(part 1 of 2)
# Autodesk Inventor assembly: Shield_99
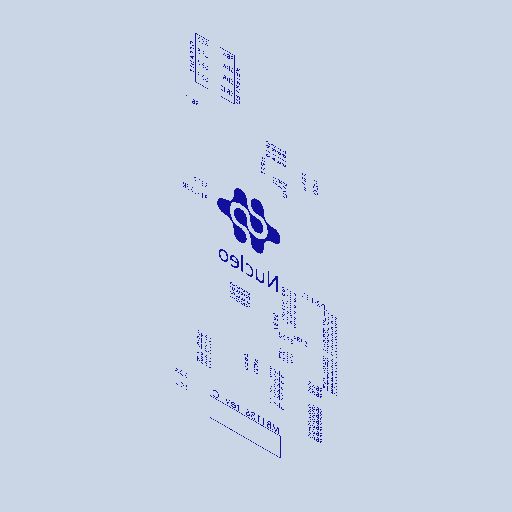
[picture p0: Inventor's stored thumbnail of the model, 512x512]
Saved by Autodesk Inventor 2022 (Build 260153000, 153)
## iProperties
Created: 2022-03-24
Part Number: Shield_99
Document SubType Name: Assembly
Designer: dvorakj
Author: dvorakj
## Documents named in this file (319)
- C:\Users\dvorakj\Documents\Inventor\Bakalarka\altium export\Shield_99.iam
- C:\Users\dvorakj\Documents\Inventor\Bakalarka\altium export\NUCLEO-F411RE_PCB_BOTTOM_Overlay_Varsay_X_8Dlan.ipt
- C:\Users\dvorakj\Documents\Inventor\Bakalarka\altium export\NUCLEO-F411RE_PCB_BOTTOM_Overlay_Varsay_X_8Dlan_1.ipt
- C:\Users\dvorakj\Documents\Inventor\Bakalarka\altium export\NUCLEO-F411RE_PCB_BOTTOM_Overlay_Varsay_X_8Dlan_2.ipt
- C:\Users\dvorakj\Documents\Inventor\Bakalarka\altium export\NUCLEO-F411RE_PCB_BOTTOM_Overlay_Varsay_X_8Dlan_3.ipt
- C:\Users\dvorakj\Documents\Inventor\Bakalarka\altium export\NUCLEO-F411RE_PCB_BOTTOM_Overlay_Varsay_X_8Dlan_4.ipt
- C:\Users\dvorakj\Documents\Inventor\Bakalarka\altium export\NUCLEO-F411RE_PCB_BOTTOM_Overlay_Varsay_X_8Dlan_5.ipt
- C:\Users\dvorakj\Documents\Inventor\Bakalarka\altium export\NUCLEO-F411RE_PCB_BOTTOM_Overlay_Varsay_X_8Dlan_6.ipt
- C:\Users\dvorakj\Documents\Inventor\Bakalarka\altium export\NUCLEO-F411RE_PCB_BOTTOM_Overlay_Varsay_X_8Dlan_7.ipt
- C:\Users\dvorakj\Documents\Inventor\Bakalarka\altium export\NUCLEO-F411RE_PCB_BOTTOM_Overlay_Varsay_X_8Dlan_8.ipt
- C:\Users\dvorakj\Documents\Inventor\Bakalarka\altium export\NUCLEO-F411RE_PCB_BOTTOM_Overlay_Varsay_X_8Dlan_9.ipt
- C:\Users\dvorakj\Documents\Inventor\Bakalarka\altium export\NUCLEO-F411RE_PCB_BOTTOM_Overlay_Varsay_X_8Dlan_10.ipt
- C:\Users\dvorakj\Documents\Inventor\Bakalarka\altium export\NUCLEO-F411RE_PCB_BOTTOM_Overlay_Varsay_X_8Dlan_11.ipt
- C:\Users\dvorakj\Documents\Inventor\Bakalarka\altium export\NUCLEO-F411RE_PCB_BOTTOM_Overlay_Varsay_X_8Dlan_12.ipt
- C:\Users\dvorakj\Documents\Inventor\Bakalarka\altium export\NUCLEO-F411RE_PCB_BOTTOM_Overlay_Varsay_X_8Dlan_13.ipt
- C:\Users\dvorakj\Documents\Inventor\Bakalarka\altium export\NUCLEO-F411RE_PCB_BOTTOM_Overlay_Varsay_X_8Dlan_14.ipt
- C:\Users\dvorakj\Documents\Inventor\Bakalarka\altium export\NUCLEO-F411RE_PCB_BOTTOM_Overlay_Varsay_X_8Dlan_15.ipt
- C:\Users\dvorakj\Documents\Inventor\Bakalarka\altium export\NUCLEO-F411RE_PCB_BOTTOM_Overlay_Varsay_X_8Dlan_16.ipt
- C:\Users\dvorakj\Documents\Inventor\Bakalarka\altium export\NUCLEO-F411RE_PCB_BOTTOM_Overlay_Varsay_X_8Dlan_17.ipt
- C:\Users\dvorakj\Documents\Inventor\Bakalarka\altium export\NUCLEO-F411RE_PCB_BOTTOM_Overlay_Varsay_X_8Dlan_18.ipt
- C:\Users\dvorakj\Documents\Inventor\Bakalarka\altium export\NUCLEO-F411RE_PCB_BOTTOM_Overlay_Varsay_X_8Dlan_19.ipt
- C:\Users\dvorakj\Documents\Inventor\Bakalarka\altium export\NUCLEO-F411RE_PCB_BOTTOM_Overlay_Varsay_X_8Dlan_20.ipt
- C:\Users\dvorakj\Documents\Inventor\Bakalarka\altium export\NUCLEO-F411RE_PCB_BOTTOM_Overlay_Varsay_X_8Dlan_21.ipt
- C:\Users\dvorakj\Documents\Inventor\Bakalarka\altium export\NUCLEO-F411RE_PCB_BOTTOM_Overlay_Varsay_X_8Dlan_22.ipt
- C:\Users\dvorakj\Documents\Inventor\Bakalarka\altium export\NUCLEO-F411RE_PCB_BOTTOM_Overlay_Varsay_X_8Dlan_23.ipt
- C:\Users\dvorakj\Documents\Inventor\Bakalarka\altium export\NUCLEO-F411RE_PCB_BOTTOM_Overlay_Varsay_X_8Dlan_24.ipt
- C:\Users\dvorakj\Documents\Inventor\Bakalarka\altium export\NUCLEO-F411RE_PCB_BOTTOM_Overlay_Varsay_X_8Dlan_25.ipt
- C:\Users\dvorakj\Documents\Inventor\Bakalarka\altium export\NUCLEO-F411RE_PCB_BOTTOM_Overlay_Varsay_X_8Dlan_26.ipt
- C:\Users\dvorakj\Documents\Inventor\Bakalarka\altium export\NUCLEO-F411RE_PCB_BOTTOM_Overlay_Varsay_X_8Dlan_27.ipt
- C:\Users\dvorakj\Documents\Inventor\Bakalarka\altium export\NUCLEO-F411RE_PCB_BOTTOM_Overlay_Varsay_X_8Dlan_28.ipt
- C:\Users\dvorakj\Documents\Inventor\Bakalarka\altium export\NUCLEO-F411RE_PCB_BOTTOM_Overlay_Varsay_X_8Dlan_29.ipt
- C:\Users\dvorakj\Documents\Inventor\Bakalarka\altium export\NUCLEO-F411RE_PCB_BOTTOM_Overlay_Varsay_X_8Dlan_30.ipt
- C:\Users\dvorakj\Documents\Inventor\Bakalarka\altium export\NUCLEO-F411RE_PCB_BOTTOM_Overlay_Varsay_X_8Dlan_31.ipt
- C:\Users\dvorakj\Documents\Inventor\Bakalarka\altium export\NUCLEO-F411RE_PCB_BOTTOM_Overlay_Varsay_X_8Dlan_32.ipt
- C:\Users\dvorakj\Documents\Inventor\Bakalarka\altium export\NUCLEO-F411RE_PCB_BOTTOM_Overlay_Varsay_X_8Dlan_33.ipt
- C:\Users\dvorakj\Documents\Inventor\Bakalarka\altium export\NUCLEO-F411RE_PCB_BOTTOM_Overlay_Varsay_X_8Dlan_34.ipt
- C:\Users\dvorakj\Documents\Inventor\Bakalarka\altium export\NUCLEO-F411RE_PCB_BOTTOM_Overlay_Varsay_X_8Dlan_35.ipt
- C:\Users\dvorakj\Documents\Inventor\Bakalarka\altium export\NUCLEO-F411RE_PCB_BOTTOM_Overlay_Varsay_X_8Dlan_36.ipt
- C:\Users\dvorakj\Documents\Inventor\Bakalarka\altium export\NUCLEO-F411RE_PCB_BOTTOM_Overlay_Varsay_X_8Dlan_37.ipt
- C:\Users\dvorakj\Documents\Inventor\Bakalarka\altium export\NUCLEO-F411RE_PCB_BOTTOM_Overlay_Varsay_X_8Dlan_38.ipt
- C:\Users\dvorakj\Documents\Inventor\Bakalarka\altium export\NUCLEO-F411RE_PCB_BOTTOM_Overlay_Varsay_X_8Dlan_39.ipt
- C:\Users\dvorakj\Documents\Inventor\Bakalarka\altium export\NUCLEO-F411RE_PCB_BOTTOM_Overlay_Varsay_X_8Dlan_40.ipt
- C:\Users\dvorakj\Documents\Inventor\Bakalarka\altium export\NUCLEO-F411RE_PCB_BOTTOM_Overlay_Varsay_X_8Dlan_41.ipt
- C:\Users\dvorakj\Documents\Inventor\Bakalarka\altium export\NUCLEO-F411RE_PCB_BOTTOM_Overlay_Varsay_X_8Dlan_42.ipt
- C:\Users\dvorakj\Documents\Inventor\Bakalarka\altium export\NUCLEO-F411RE_PCB_BOTTOM_Overlay_Varsay_X_8Dlan_43.ipt
- C:\Users\dvorakj\Documents\Inventor\Bakalarka\altium export\NUCLEO-F411RE_PCB_BOTTOM_Overlay_Varsay_X_8Dlan_44.ipt
- C:\Users\dvorakj\Documents\Inventor\Bakalarka\altium export\NUCLEO-F411RE_PCB_BOTTOM_Overlay_Varsay_X_8Dlan_45.ipt
- C:\Users\dvorakj\Documents\Inventor\Bakalarka\altium export\NUCLEO-F411RE_PCB_BOTTOM_Overlay_Varsay_X_8Dlan_46.ipt
- C:\Users\dvorakj\Documents\Inventor\Bakalarka\altium export\NUCLEO-F411RE_PCB_BOTTOM_Overlay_Varsay_X_8Dlan_47.ipt
- C:\Users\dvorakj\Documents\Inventor\Bakalarka\altium export\NUCLEO-F411RE_PCB_BOTTOM_Overlay_Varsay_X_8Dlan_48.ipt
- C:\Users\dvorakj\Documents\Inventor\Bakalarka\altium export\NUCLEO-F411RE_PCB_BOTTOM_Overlay_Varsay_X_8Dlan_49.ipt
- C:\Users\dvorakj\Documents\Inventor\Bakalarka\altium export\NUCLEO-F411RE_PCB_BOTTOM_Overlay_Varsay_X_8Dlan_50.ipt
- C:\Users\dvorakj\Documents\Inventor\Bakalarka\altium export\NUCLEO-F411RE_PCB_BOTTOM_Overlay_Varsay_X_8Dlan_51.ipt
- C:\Users\dvorakj\Documents\Inventor\Bakalarka\altium export\NUCLEO-F411RE_PCB_BOTTOM_Overlay_Varsay_X_8Dlan_52.ipt
- C:\Users\dvorakj\Documents\Inventor\Bakalarka\altium export\NUCLEO-F411RE_PCB_BOTTOM_Overlay_Varsay_X_8Dlan_53.ipt
- C:\Users\dvorakj\Documents\Inventor\Bakalarka\altium export\NUCLEO-F411RE_PCB_BOTTOM_Overlay_Varsay_X_8Dlan_54.ipt
- C:\Users\dvorakj\Documents\Inventor\Bakalarka\altium export\NUCLEO-F411RE_PCB_BOTTOM_Overlay_Varsay_X_8Dlan_55.ipt
- C:\Users\dvorakj\Documents\Inventor\Bakalarka\altium export\NUCLEO-F411RE_PCB_BOTTOM_Overlay_Varsay_X_8Dlan_56.ipt
- C:\Users\dvorakj\Documents\Inventor\Bakalarka\altium export\NUCLEO-F411RE_PCB_BOTTOM_Overlay_Varsay_X_8Dlan_57.ipt
- C:\Users\dvorakj\Documents\Inventor\Bakalarka\altium export\NUCLEO-F411RE_PCB_BOTTOM_Overlay_Varsay_X_8Dlan_58.ipt
- C:\Users\dvorakj\Documents\Inventor\Bakalarka\altium export\NUCLEO-F411RE_PCB_BOTTOM_Overlay_Varsay_X_8Dlan_59.ipt
- C:\Users\dvorakj\Documents\Inventor\Bakalarka\altium export\NUCLEO-F411RE_PCB_BOTTOM_Overlay_Varsay_X_8Dlan_60.ipt
- C:\Users\dvorakj\Documents\Inventor\Bakalarka\altium export\NUCLEO-F411RE_PCB_BOTTOM_Overlay_Varsay_X_8Dlan_61.ipt
- C:\Users\dvorakj\Documents\Inventor\Bakalarka\altium export\NUCLEO-F411RE_PCB_BOTTOM_Overlay_Varsay_X_8Dlan_62.ipt
- C:\Users\dvorakj\Documents\Inventor\Bakalarka\altium export\NUCLEO-F411RE_PCB_BOTTOM_Overlay_Varsay_X_8Dlan_63.ipt
- C:\Users\dvorakj\Documents\Inventor\Bakalarka\altium export\NUCLEO-F411RE_PCB_BOTTOM_Overlay_Varsay_X_8Dlan_64.ipt
- C:\Users\dvorakj\Documents\Inventor\Bakalarka\altium export\NUCLEO-F411RE_PCB_BOTTOM_Overlay_Varsay_X_8Dlan_65.ipt
- C:\Users\dvorakj\Documents\Inventor\Bakalarka\altium export\NUCLEO-F411RE_PCB_BOTTOM_Overlay_Varsay_X_8Dlan_66.ipt
- C:\Users\dvorakj\Documents\Inventor\Bakalarka\altium export\NUCLEO-F411RE_PCB_BOTTOM_Overlay_Varsay_X_8Dlan_67.ipt
- C:\Users\dvorakj\Documents\Inventor\Bakalarka\altium export\NUCLEO-F411RE_PCB_BOTTOM_Overlay_Varsay_X_8Dlan_68.ipt
- C:\Users\dvorakj\Documents\Inventor\Bakalarka\altium export\NUCLEO-F411RE_PCB_BOTTOM_Overlay_Varsay_X_8Dlan_69.ipt
- C:\Users\dvorakj\Documents\Inventor\Bakalarka\altium export\NUCLEO-F411RE_PCB_BOTTOM_Overlay_Varsay_X_8Dlan_70.ipt
- C:\Users\dvorakj\Documents\Inventor\Bakalarka\altium export\NUCLEO-F411RE_PCB_BOTTOM_Overlay_Varsay_X_8Dlan_71.ipt
- C:\Users\dvorakj\Documents\Inventor\Bakalarka\altium export\NUCLEO-F411RE_PCB_BOTTOM_Overlay_Varsay_X_8Dlan_72.ipt
- C:\Users\dvorakj\Documents\Inventor\Bakalarka\altium export\NUCLEO-F411RE_PCB_BOTTOM_Overlay_Varsay_X_8Dlan_73.ipt
- C:\Users\dvorakj\Documents\Inventor\Bakalarka\altium export\NUCLEO-F411RE_PCB_BOTTOM_Overlay_Varsay_X_8Dlan_74.ipt
- C:\Users\dvorakj\Documents\Inventor\Bakalarka\altium export\NUCLEO-F411RE_PCB_BOTTOM_Overlay_Varsay_X_8Dlan_75.ipt
- C:\Users\dvorakj\Documents\Inventor\Bakalarka\altium export\NUCLEO-F411RE_PCB_BOTTOM_Overlay_Varsay_X_8Dlan_76.ipt
- C:\Users\dvorakj\Documents\Inventor\Bakalarka\altium export\NUCLEO-F411RE_PCB_BOTTOM_Overlay_Varsay_X_8Dlan_77.ipt
- C:\Users\dvorakj\Documents\Inventor\Bakalarka\altium export\NUCLEO-F411RE_PCB_BOTTOM_Overlay_Varsay_X_8Dlan_78.ipt
- C:\Users\dvorakj\Documents\Inventor\Bakalarka\altium export\NUCLEO-F411RE_PCB_BOTTOM_Overlay_Varsay_X_8Dlan_79.ipt
- C:\Users\dvorakj\Documents\Inventor\Bakalarka\altium export\NUCLEO-F411RE_PCB_BOTTOM_Overlay_Varsay_X_8Dlan_80.ipt
- C:\Users\dvorakj\Documents\Inventor\Bakalarka\altium export\NUCLEO-F411RE_PCB_BOTTOM_Overlay_Varsay_X_8Dlan_81.ipt
- C:\Users\dvorakj\Documents\Inventor\Bakalarka\altium export\NUCLEO-F411RE_PCB_BOTTOM_Overlay_Varsay_X_8Dlan_82.ipt
- C:\Users\dvorakj\Documents\Inventor\Bakalarka\altium export\NUCLEO-F411RE_PCB_BOTTOM_Overlay_Varsay_X_8Dlan_83.ipt
- C:\Users\dvorakj\Documents\Inventor\Bakalarka\altium export\NUCLEO-F411RE_PCB_BOTTOM_Overlay_Varsay_X_8Dlan_84.ipt
- C:\Users\dvorakj\Documents\Inventor\Bakalarka\altium export\NUCLEO-F411RE_PCB_BOTTOM_Overlay_Varsay_X_8Dlan_85.ipt
- C:\Users\dvorakj\Documents\Inventor\Bakalarka\altium export\NUCLEO-F411RE_PCB_BOTTOM_Overlay_Varsay_X_8Dlan_86.ipt
- C:\Users\dvorakj\Documents\Inventor\Bakalarka\altium export\NUCLEO-F411RE_PCB_BOTTOM_Overlay_Varsay_X_8Dlan_87.ipt
- C:\Users\dvorakj\Documents\Inventor\Bakalarka\altium export\NUCLEO-F411RE_PCB_BOTTOM_Overlay_Varsay_X_8Dlan_88.ipt
- C:\Users\dvorakj\Documents\Inventor\Bakalarka\altium export\NUCLEO-F411RE_PCB_BOTTOM_Overlay_Varsay_X_8Dlan_89.ipt
- C:\Users\dvorakj\Documents\Inventor\Bakalarka\altium export\NUCLEO-F411RE_PCB_BOTTOM_Overlay_Varsay_X_8Dlan_90.ipt
- C:\Users\dvorakj\Documents\Inventor\Bakalarka\altium export\NUCLEO-F411RE_PCB_BOTTOM_Overlay_Varsay_X_8Dlan_91.ipt
- C:\Users\dvorakj\Documents\Inventor\Bakalarka\altium export\NUCLEO-F411RE_PCB_BOTTOM_Overlay_Varsay_X_8Dlan_92.ipt
- C:\Users\dvorakj\Documents\Inventor\Bakalarka\altium export\NUCLEO-F411RE_PCB_BOTTOM_Overlay_Varsay_X_8Dlan_93.ipt
- C:\Users\dvorakj\Documents\Inventor\Bakalarka\altium export\NUCLEO-F411RE_PCB_BOTTOM_Overlay_Varsay_X_8Dlan_94.ipt
- C:\Users\dvorakj\Documents\Inventor\Bakalarka\altium export\NUCLEO-F411RE_PCB_BOTTOM_Overlay_Varsay_X_8Dlan_95.ipt
- C:\Users\dvorakj\Documents\Inventor\Bakalarka\altium export\NUCLEO-F411RE_PCB_BOTTOM_Overlay_Varsay_X_8Dlan_96.ipt
- C:\Users\dvorakj\Documents\Inventor\Bakalarka\altium export\NUCLEO-F411RE_PCB_BOTTOM_Overlay_Varsay_X_8Dlan_97.ipt
- C:\Users\dvorakj\Documents\Inventor\Bakalarka\altium export\NUCLEO-F411RE_PCB_BOTTOM_Overlay_Varsay_X_8Dlan_98.ipt
- C:\Users\dvorakj\Documents\Inventor\Bakalarka\altium export\NUCLEO-F411RE_PCB_BOTTOM_Overlay_Varsay_X_8Dlan_99.ipt
- C:\Users\dvorakj\Documents\Inventor\Bakalarka\altium export\NUCLEO-F411RE_PCB_BOTTOM_Overlay_Varsay_X_8Dlan_100.ipt
- C:\Users\dvorakj\Documents\Inventor\Bakalarka\altium export\NUCLEO-F411RE_PCB_BOTTOM_Overlay_Varsay_X_8Dlan_101.ipt
- C:\Users\dvorakj\Documents\Inventor\Bakalarka\altium export\NUCLEO-F411RE_PCB_BOTTOM_Overlay_Varsay_X_8Dlan_102.ipt
- C:\Users\dvorakj\Documents\Inventor\Bakalarka\altium export\NUCLEO-F411RE_PCB_BOTTOM_Overlay_Varsay_X_8Dlan_103.ipt
- C:\Users\dvorakj\Documents\Inventor\Bakalarka\altium export\NUCLEO-F411RE_PCB_BOTTOM_Overlay_Varsay_X_8Dlan_104.ipt
- C:\Users\dvorakj\Documents\Inventor\Bakalarka\altium export\NUCLEO-F411RE_PCB_BOTTOM_Overlay_Varsay_X_8Dlan_105.ipt
- C:\Users\dvorakj\Documents\Inventor\Bakalarka\altium export\NUCLEO-F411RE_PCB_BOTTOM_Overlay_Varsay_X_8Dlan_106.ipt
- C:\Users\dvorakj\Documents\Inventor\Bakalarka\altium export\NUCLEO-F411RE_PCB_BOTTOM_Overlay_Varsay_X_8Dlan_107.ipt
- C:\Users\dvorakj\Documents\Inventor\Bakalarka\altium export\NUCLEO-F411RE_PCB_BOTTOM_Overlay_Varsay_X_8Dlan_108.ipt
- C:\Users\dvorakj\Documents\Inventor\Bakalarka\altium export\NUCLEO-F411RE_PCB_BOTTOM_Overlay_Varsay_X_8Dlan_109.ipt
- C:\Users\dvorakj\Documents\Inventor\Bakalarka\altium export\NUCLEO-F411RE_PCB_BOTTOM_Overlay_Varsay_X_8Dlan_110.ipt
- C:\Users\dvorakj\Documents\Inventor\Bakalarka\altium export\NUCLEO-F411RE_PCB_BOTTOM_Overlay_Varsay_X_8Dlan_111.ipt
- C:\Users\dvorakj\Documents\Inventor\Bakalarka\altium export\NUCLEO-F411RE_PCB_BOTTOM_Overlay_Varsay_X_8Dlan_112.ipt
- C:\Users\dvorakj\Documents\Inventor\Bakalarka\altium export\NUCLEO-F411RE_PCB_BOTTOM_Overlay_Varsay_X_8Dlan_113.ipt
- C:\Users\dvorakj\Documents\Inventor\Bakalarka\altium export\NUCLEO-F411RE_PCB_BOTTOM_Overlay_Varsay_X_8Dlan_114.ipt
- C:\Users\dvorakj\Documents\Inventor\Bakalarka\altium export\NUCLEO-F411RE_PCB_BOTTOM_Overlay_Varsay_X_8Dlan_115.ipt
- C:\Users\dvorakj\Documents\Inventor\Bakalarka\altium export\NUCLEO-F411RE_PCB_BOTTOM_Overlay_Varsay_X_8Dlan_116.ipt
- C:\Users\dvorakj\Documents\Inventor\Bakalarka\altium export\NUCLEO-F411RE_PCB_BOTTOM_Overlay_Varsay_X_8Dlan_117.ipt
- C:\Users\dvorakj\Documents\Inventor\Bakalarka\altium export\NUCLEO-F411RE_PCB_BOTTOM_Overlay_Varsay_X_8Dlan_118.ipt
- C:\Users\dvorakj\Documents\Inventor\Bakalarka\altium export\NUCLEO-F411RE_PCB_BOTTOM_Overlay_Varsay_X_8Dlan_119.ipt
- C:\Users\dvorakj\Documents\Inventor\Bakalarka\altium export\NUCLEO-F411RE_PCB_BOTTOM_Overlay_Varsay_X_8Dlan_120.ipt
- C:\Users\dvorakj\Documents\Inventor\Bakalarka\altium export\NUCLEO-F411RE_PCB_BOTTOM_Overlay_Varsay_X_8Dlan_121.ipt
- C:\Users\dvorakj\Documents\Inventor\Bakalarka\altium export\NUCLEO-F411RE_PCB_BOTTOM_Overlay_Varsay_X_8Dlan_122.ipt
- C:\Users\dvorakj\Documents\Inventor\Bakalarka\altium export\NUCLEO-F411RE_PCB_BOTTOM_Overlay_Varsay_X_8Dlan_123.ipt
- C:\Users\dvorakj\Documents\Inventor\Bakalarka\altium export\NUCLEO-F411RE_PCB_BOTTOM_Overlay_Varsay_X_8Dlan_124.ipt
- C:\Users\dvorakj\Documents\Inventor\Bakalarka\altium export\NUCLEO-F411RE_PCB_BOTTOM_Overlay_Varsay_X_8Dlan_125.ipt
- C:\Users\dvorakj\Documents\Inventor\Bakalarka\altium export\NUCLEO-F411RE_PCB_BOTTOM_Overlay_Varsay_X_8Dlan_126.ipt
- C:\Users\dvorakj\Documents\Inventor\Bakalarka\altium export\NUCLEO-F411RE_PCB_BOTTOM_Overlay_Varsay_X_8Dlan_127.ipt
- C:\Users\dvorakj\Documents\Inventor\Bakalarka\altium export\NUCLEO-F411RE_PCB_BOTTOM_Overlay_Varsay_X_8Dlan_128.ipt
- C:\Users\dvorakj\Documents\Inventor\Bakalarka\altium export\NUCLEO-F411RE_PCB_BOTTOM_Overlay_Varsay_X_8Dlan_129.ipt
- C:\Users\dvorakj\Documents\Inventor\Bakalarka\altium export\NUCLEO-F411RE_PCB_BOTTOM_Overlay_Varsay_X_8Dlan_130.ipt
- C:\Users\dvorakj\Documents\Inventor\Bakalarka\altium export\NUCLEO-F411RE_PCB_BOTTOM_Overlay_Varsay_X_8Dlan_131.ipt
- C:\Users\dvorakj\Documents\Inventor\Bakalarka\altium export\NUCLEO-F411RE_PCB_BOTTOM_Overlay_Varsay_X_8Dlan_132.ipt
- C:\Users\dvorakj\Documents\Inventor\Bakalarka\altium export\NUCLEO-F411RE_PCB_BOTTOM_Overlay_Varsay_X_8Dlan_133.ipt
- C:\Users\dvorakj\Documents\Inventor\Bakalarka\altium export\NUCLEO-F411RE_PCB_BOTTOM_Overlay_Varsay_X_8Dlan_134.ipt
- C:\Users\dvorakj\Documents\Inventor\Bakalarka\altium export\NUCLEO-F411RE_PCB_BOTTOM_Overlay_Varsay_X_8Dlan_135.ipt
- C:\Users\dvorakj\Documents\Inventor\Bakalarka\altium export\NUCLEO-F411RE_PCB_BOTTOM_Overlay_Varsay_X_8Dlan_136.ipt
- C:\Users\dvorakj\Documents\Inventor\Bakalarka\altium export\NUCLEO-F411RE_PCB_BOTTOM_Overlay_Varsay_X_8Dlan_137.ipt
- C:\Users\dvorakj\Documents\Inventor\Bakalarka\altium export\NUCLEO-F411RE_PCB_BOTTOM_Overlay_Varsay_X_8Dlan_138.ipt
- C:\Users\dvorakj\Documents\Inventor\Bakalarka\altium export\NUCLEO-F411RE_PCB_BOTTOM_Overlay_Varsay_X_8Dlan_139.ipt
- C:\Users\dvorakj\Documents\Inventor\Bakalarka\altium export\NUCLEO-F411RE_PCB_BOTTOM_Overlay_Varsay_X_8Dlan_140.ipt
- C:\Users\dvorakj\Documents\Inventor\Bakalarka\altium export\NUCLEO-F411RE_PCB_BOTTOM_Overlay_Varsay_X_8Dlan_141.ipt
- C:\Users\dvorakj\Documents\Inventor\Bakalarka\altium export\NUCLEO-F411RE_PCB_BOTTOM_Overlay_Varsay_X_8Dlan_142.ipt
- C:\Users\dvorakj\Documents\Inventor\Bakalarka\altium export\NUCLEO-F411RE_PCB_BOTTOM_Overlay_Varsay_X_8Dlan_143.ipt
- C:\Users\dvorakj\Documents\Inventor\Bakalarka\altium export\NUCLEO-F411RE_PCB_BOTTOM_Overlay_Varsay_X_8Dlan_144.ipt
- C:\Users\dvorakj\Documents\Inventor\Bakalarka\altium export\NUCLEO-F411RE_PCB_BOTTOM_Overlay_Varsay_X_8Dlan_145.ipt
- C:\Users\dvorakj\Documents\Inventor\Bakalarka\altium export\NUCLEO-F411RE_PCB_BOTTOM_Overlay_Varsay_X_8Dlan_146.ipt
- C:\Users\dvorakj\Documents\Inventor\Bakalarka\altium export\NUCLEO-F411RE_PCB_BOTTOM_Overlay_Varsay_X_8Dlan_147.ipt
- C:\Users\dvorakj\Documents\Inventor\Bakalarka\altium export\NUCLEO-F411RE_PCB_BOTTOM_Overlay_Varsay_X_8Dlan_148.ipt
- C:\Users\dvorakj\Documents\Inventor\Bakalarka\altium export\NUCLEO-F411RE_PCB_BOTTOM_Overlay_Varsay_X_8Dlan_149.ipt
- C:\Users\dvorakj\Documents\Inventor\Bakalarka\altium export\NUCLEO-F411RE_PCB_BOTTOM_Overlay_Varsay_X_8Dlan_150.ipt
- C:\Users\dvorakj\Documents\Inventor\Bakalarka\altium export\NUCLEO-F411RE_PCB_BOTTOM_Overlay_Varsay_X_8Dlan_151.ipt
- C:\Users\dvorakj\Documents\Inventor\Bakalarka\altium export\NUCLEO-F411RE_PCB_BOTTOM_Overlay_Varsay_X_8Dlan_152.ipt
- C:\Users\dvorakj\Documents\Inventor\Bakalarka\altium export\NUCLEO-F411RE_PCB_BOTTOM_Overlay_Varsay_X_8Dlan_153.ipt
- C:\Users\dvorakj\Documents\Inventor\Bakalarka\altium export\NUCLEO-F411RE_PCB_BOTTOM_Overlay_Varsay_X_8Dlan_154.ipt
- C:\Users\dvorakj\Documents\Inventor\Bakalarka\altium export\NUCLEO-F411RE_PCB_BOTTOM_Overlay_Varsay_X_8Dlan_155.ipt
- C:\Users\dvorakj\Documents\Inventor\Bakalarka\altium export\NUCLEO-F411RE_PCB_BOTTOM_Overlay_Varsay_X_8Dlan_156.ipt
- C:\Users\dvorakj\Documents\Inventor\Bakalarka\altium export\NUCLEO-F411RE_PCB_BOTTOM_Overlay_Varsay_X_8Dlan_157.ipt
- C:\Users\dvorakj\Documents\Inventor\Bakalarka\altium export\NUCLEO-F411RE_PCB_BOTTOM_Overlay_Varsay_X_8Dlan_158.ipt
- C:\Users\dvorakj\Documents\Inventor\Bakalarka\altium export\NUCLEO-F411RE_PCB_BOTTOM_Overlay_Varsay_X_8Dlan_159.ipt
- C:\Users\dvorakj\Documents\Inventor\Bakalarka\altium export\NUCLEO-F411RE_PCB_BOTTOM_Overlay_Varsay_X_8Dlan_160.ipt
- C:\Users\dvorakj\Documents\Inventor\Bakalarka\altium export\NUCLEO-F411RE_PCB_BOTTOM_Overlay_Varsay_X_8Dlan_161.ipt
- C:\Users\dvorakj\Documents\Inventor\Bakalarka\altium export\NUCLEO-F411RE_PCB_BOTTOM_Overlay_Varsay_X_8Dlan_162.ipt
- C:\Users\dvorakj\Documents\Inventor\Bakalarka\altium export\NUCLEO-F411RE_PCB_BOTTOM_Overlay_Varsay_X_8Dlan_163.ipt
- C:\Users\dvorakj\Documents\Inventor\Bakalarka\altium export\NUCLEO-F411RE_PCB_BOTTOM_Overlay_Varsay_X_8Dlan_164.ipt
- C:\Users\dvorakj\Documents\Inventor\Bakalarka\altium export\NUCLEO-F411RE_PCB_BOTTOM_Overlay_Varsay_X_8Dlan_165.ipt
- C:\Users\dvorakj\Documents\Inventor\Bakalarka\altium export\NUCLEO-F411RE_PCB_BOTTOM_Overlay_Varsay_X_8Dlan_166.ipt
- C:\Users\dvorakj\Documents\Inventor\Bakalarka\altium export\NUCLEO-F411RE_PCB_BOTTOM_Overlay_Varsay_X_8Dlan_167.ipt
- C:\Users\dvorakj\Documents\Inventor\Bakalarka\altium export\NUCLEO-F411RE_PCB_BOTTOM_Overlay_Varsay_X_8Dlan_168.ipt
- C:\Users\dvorakj\Documents\Inventor\Bakalarka\altium export\NUCLEO-F411RE_PCB_BOTTOM_Overlay_Varsay_X_8Dlan_169.ipt
- C:\Users\dvorakj\Documents\Inventor\Bakalarka\altium export\NUCLEO-F411RE_PCB_BOTTOM_Overlay_Varsay_X_8Dlan_170.ipt
- C:\Users\dvorakj\Documents\Inventor\Bakalarka\altium export\NUCLEO-F411RE_PCB_BOTTOM_Overlay_Varsay_X_8Dlan_171.ipt
- C:\Users\dvorakj\Documents\Inventor\Bakalarka\altium export\NUCLEO-F411RE_PCB_BOTTOM_Overlay_Varsay_X_8Dlan_172.ipt
- C:\Users\dvorakj\Documents\Inventor\Bakalarka\altium export\NUCLEO-F411RE_PCB_BOTTOM_Overlay_Varsay_X_8Dlan_173.ipt
- C:\Users\dvorakj\Documents\Inventor\Bakalarka\altium export\NUCLEO-F411RE_PCB_BOTTOM_Overlay_Varsay_X_8Dlan_174.ipt
- C:\Users\dvorakj\Documents\Inventor\Bakalarka\altium export\NUCLEO-F411RE_PCB_BOTTOM_Overlay_Varsay_X_8Dlan_175.ipt
- C:\Users\dvorakj\Documents\Inventor\Bakalarka\altium export\NUCLEO-F411RE_PCB_BOTTOM_Overlay_Varsay_X_8Dlan_176.ipt
- C:\Users\dvorakj\Documents\Inventor\Bakalarka\altium export\NUCLEO-F411RE_PCB_BOTTOM_Overlay_Varsay_X_8Dlan_177.ipt
- C:\Users\dvorakj\Documents\Inventor\Bakalarka\altium export\NUCLEO-F411RE_PCB_BOTTOM_Overlay_Varsay_X_8Dlan_178.ipt
- C:\Users\dvorakj\Documents\Inventor\Bakalarka\altium export\NUCLEO-F411RE_PCB_BOTTOM_Overlay_Varsay_X_8Dlan_179.ipt
- C:\Users\dvorakj\Documents\Inventor\Bakalarka\altium export\NUCLEO-F411RE_PCB_BOTTOM_Overlay_Varsay_X_8Dlan_180.ipt
- C:\Users\dvorakj\Documents\Inventor\Bakalarka\altium export\NUCLEO-F411RE_PCB_BOTTOM_Overlay_Varsay_X_8Dlan_181.ipt
- C:\Users\dvorakj\Documents\Inventor\Bakalarka\altium export\NUCLEO-F411RE_PCB_BOTTOM_Overlay_Varsay_X_8Dlan_182.ipt
- C:\Users\dvorakj\Documents\Inventor\Bakalarka\altium export\NUCLEO-F411RE_PCB_BOTTOM_Overlay_Varsay_X_8Dlan_183.ipt
- C:\Users\dvorakj\Documents\Inventor\Bakalarka\altium export\NUCLEO-F411RE_PCB_BOTTOM_Overlay_Varsay_X_8Dlan_184.ipt
- C:\Users\dvorakj\Documents\Inventor\Bakalarka\altium export\NUCLEO-F411RE_PCB_BOTTOM_Overlay_Varsay_X_8Dlan_185.ipt
- C:\Users\dvorakj\Documents\Inventor\Bakalarka\altium export\NUCLEO-F411RE_PCB_BOTTOM_Overlay_Varsay_X_8Dlan_186.ipt
- C:\Users\dvorakj\Documents\Inventor\Bakalarka\altium export\NUCLEO-F411RE_PCB_BOTTOM_Overlay_Varsay_X_8Dlan_187.ipt
- C:\Users\dvorakj\Documents\Inventor\Bakalarka\altium export\NUCLEO-F411RE_PCB_BOTTOM_Overlay_Varsay_X_8Dlan_188.ipt
- C:\Users\dvorakj\Documents\Inventor\Bakalarka\altium export\NUCLEO-F411RE_PCB_BOTTOM_Overlay_Varsay_X_8Dlan_189.ipt
- C:\Users\dvorakj\Documents\Inventor\Bakalarka\altium export\NUCLEO-F411RE_PCB_BOTTOM_Overlay_Varsay_X_8Dlan_190.ipt
- C:\Users\dvorakj\Documents\Inventor\Bakalarka\altium export\NUCLEO-F411RE_PCB_BOTTOM_Overlay_Varsay_X_8Dlan_191.ipt
- C:\Users\dvorakj\Documents\Inventor\Bakalarka\altium export\NUCLEO-F411RE_PCB_BOTTOM_Overlay_Varsay_X_8Dlan_192.ipt
- C:\Users\dvorakj\Documents\Inventor\Bakalarka\altium export\NUCLEO-F411RE_PCB_BOTTOM_Overlay_Varsay_X_8Dlan_193.ipt
- C:\Users\dvorakj\Documents\Inventor\Bakalarka\altium export\NUCLEO-F411RE_PCB_BOTTOM_Overlay_Varsay_X_8Dlan_194.ipt
- C:\Users\dvorakj\Documents\Inventor\Bakalarka\altium export\NUCLEO-F411RE_PCB_BOTTOM_Overlay_Varsay_X_8Dlan_195.ipt
- C:\Users\dvorakj\Documents\Inventor\Bakalarka\altium export\NUCLEO-F411RE_PCB_BOTTOM_Overlay_Varsay_X_8Dlan_196.ipt
- C:\Users\dvorakj\Documents\Inventor\Bakalarka\altium export\NUCLEO-F411RE_PCB_BOTTOM_Overlay_Varsay_X_8Dlan_197.ipt
- C:\Users\dvorakj\Documents\Inventor\Bakalarka\altium export\NUCLEO-F411RE_PCB_BOTTOM_Overlay_Varsay_X_8Dlan_198.ipt
- C:\Users\dvorakj\Documents\Inventor\Bakalarka\altium export\NUCLEO-F411RE_PCB_BOTTOM_Overlay_Varsay_X_8Dlan_199.ipt
- C:\Users\dvorakj\Documents\Inventor\Bakalarka\altium export\NUCLEO-F411RE_PCB_BOTTOM_Overlay_Varsay_X_8Dlan_200.ipt
- C:\Users\dvorakj\Documents\Inventor\Bakalarka\altium export\NUCLEO-F411RE_PCB_BOTTOM_Overlay_Varsay_X_8Dlan_201.ipt
- C:\Users\dvorakj\Documents\Inventor\Bakalarka\altium export\NUCLEO-F411RE_PCB_BOTTOM_Overlay_Varsay_X_8Dlan_202.ipt
- C:\Users\dvorakj\Documents\Inventor\Bakalarka\altium export\NUCLEO-F411RE_PCB_BOTTOM_Overlay_Varsay_X_8Dlan_203.ipt
- C:\Users\dvorakj\Documents\Inventor\Bakalarka\altium export\NUCLEO-F411RE_PCB_BOTTOM_Overlay_Varsay_X_8Dlan_204.ipt
- C:\Users\dvorakj\Documents\Inventor\Bakalarka\altium export\NUCLEO-F411RE_PCB_BOTTOM_Overlay_Varsay_X_8Dlan_205.ipt
- C:\Users\dvorakj\Documents\Inventor\Bakalarka\altium export\NUCLEO-F411RE_PCB_BOTTOM_Overlay_Varsay_X_8Dlan_206.ipt
- C:\Users\dvorakj\Documents\Inventor\Bakalarka\altium export\NUCLEO-F411RE_PCB_BOTTOM_Overlay_Varsay_X_8Dlan_207.ipt
- C:\Users\dvorakj\Documents\Inventor\Bakalarka\altium export\NUCLEO-F411RE_PCB_BOTTOM_Overlay_Varsay_X_8Dlan_208.ipt
- C:\Users\dvorakj\Documents\Inventor\Bakalarka\altium export\NUCLEO-F411RE_PCB_BOTTOM_Overlay_Varsay_X_8Dlan_209.ipt
- C:\Users\dvorakj\Documents\Inventor\Bakalarka\altium export\NUCLEO-F411RE_PCB_BOTTOM_Overlay_Varsay_X_8Dlan_210.ipt
- C:\Users\dvorakj\Documents\Inventor\Bakalarka\altium export\NUCLEO-F411RE_PCB_BOTTOM_Overlay_Varsay_X_8Dlan_211.ipt
- C:\Users\dvorakj\Documents\Inventor\Bakalarka\altium export\NUCLEO-F411RE_PCB_BOTTOM_Overlay_Varsay_X_8Dlan_212.ipt
- C:\Users\dvorakj\Documents\Inventor\Bakalarka\altium export\NUCLEO-F411RE_PCB_BOTTOM_Overlay_Varsay_X_8Dlan_213.ipt
- C:\Users\dvorakj\Documents\Inventor\Bakalarka\altium export\NUCLEO-F411RE_PCB_BOTTOM_Overlay_Varsay_X_8Dlan_214.ipt
- C:\Users\dvorakj\Documents\Inventor\Bakalarka\altium export\NUCLEO-F411RE_PCB_BOTTOM_Overlay_Varsay_X_8Dlan_215.ipt
- C:\Users\dvorakj\Documents\Inventor\Bakalarka\altium export\NUCLEO-F411RE_PCB_BOTTOM_Overlay_Varsay_X_8Dlan_216.ipt
- C:\Users\dvorakj\Documents\Inventor\Bakalarka\altium export\NUCLEO-F411RE_PCB_BOTTOM_Overlay_Varsay_X_8Dlan_217.ipt
- C:\Users\dvorakj\Documents\Inventor\Bakalarka\altium export\NUCLEO-F411RE_PCB_BOTTOM_Overlay_Varsay_X_8Dlan_218.ipt
- C:\Users\dvorakj\Documents\Inventor\Bakalarka\altium export\NUCLEO-F411RE_PCB_BOTTOM_Overlay_Varsay_X_8Dlan_219.ipt
- C:\Users\dvorakj\Documents\Inventor\Bakalarka\altium export\NUCLEO-F411RE_PCB_BOTTOM_Overlay_Varsay_X_8Dlan_220.ipt
- C:\Users\dvorakj\Documents\Inventor\Bakalarka\altium export\NUCLEO-F411RE_PCB_BOTTOM_Overlay_Varsay_X_8Dlan_221.ipt
- C:\Users\dvorakj\Documents\Inventor\Bakalarka\altium export\NUCLEO-F411RE_PCB_BOTTOM_Overlay_Varsay_X_8Dlan_222.ipt
- C:\Users\dvorakj\Documents\Inventor\Bakalarka\altium export\NUCLEO-F411RE_PCB_BOTTOM_Overlay_Varsay_X_8Dlan_223.ipt
- C:\Users\dvorakj\Documents\Inventor\Bakalarka\altium export\NUCLEO-F411RE_PCB_BOTTOM_Overlay_Varsay_X_8Dlan_224.ipt
- C:\Users\dvorakj\Documents\Inventor\Bakalarka\altium export\NUCLEO-F411RE_PCB_BOTTOM_Overlay_Varsay_X_8Dlan_225.ipt
- C:\Users\dvorakj\Documents\Inventor\Bakalarka\altium export\NUCLEO-F411RE_PCB_BOTTOM_Overlay_Varsay_X_8Dlan_226.ipt
- C:\Users\dvorakj\Documents\Inventor\Bakalarka\altium export\NUCLEO-F411RE_PCB_BOTTOM_Overlay_Varsay_X_8Dlan_227.ipt
- C:\Users\dvorakj\Documents\Inventor\Bakalarka\altium export\NUCLEO-F411RE_PCB_BOTTOM_Overlay_Varsay_X_8Dlan_228.ipt
- C:\Users\dvorakj\Documents\Inventor\Bakalarka\altium export\NUCLEO-F411RE_PCB_BOTTOM_Overlay_Varsay_X_8Dlan_229.ipt
- C:\Users\dvorakj\Documents\Inventor\Bakalarka\altium export\NUCLEO-F411RE_PCB_BOTTOM_Overlay_Varsay_X_8Dlan_230.ipt
- C:\Users\dvorakj\Documents\Inventor\Bakalarka\altium export\NUCLEO-F411RE_PCB_BOTTOM_Overlay_Varsay_X_8Dlan_231.ipt
- C:\Users\dvorakj\Documents\Inventor\Bakalarka\altium export\NUCLEO-F411RE_PCB_BOTTOM_Overlay_Varsay_X_8Dlan_232.ipt
- C:\Users\dvorakj\Documents\Inventor\Bakalarka\altium export\NUCLEO-F411RE_PCB_BOTTOM_Overlay_Varsay_X_8Dlan_233.ipt
- C:\Users\dvorakj\Documents\Inventor\Bakalarka\altium export\NUCLEO-F411RE_PCB_BOTTOM_Overlay_Varsay_X_8Dlan_234.ipt
- C:\Users\dvorakj\Documents\Inventor\Bakalarka\altium export\NUCLEO-F411RE_PCB_BOTTOM_Overlay_Varsay_X_8Dlan_235.ipt
- C:\Users\dvorakj\Documents\Inventor\Bakalarka\altium export\NUCLEO-F411RE_PCB_BOTTOM_Overlay_Varsay_X_8Dlan_236.ipt
- C:\Users\dvorakj\Documents\Inventor\Bakalarka\altium export\NUCLEO-F411RE_PCB_BOTTOM_Overlay_Varsay_X_8Dlan_237.ipt
- C:\Users\dvorakj\Documents\Inventor\Bakalarka\altium export\NUCLEO-F411RE_PCB_BOTTOM_Overlay_Varsay_X_8Dlan_238.ipt
- C:\Users\dvorakj\Documents\Inventor\Bakalarka\altium export\NUCLEO-F411RE_PCB_BOTTOM_Overlay_Varsay_X_8Dlan_239.ipt
- C:\Users\dvorakj\Documents\Inventor\Bakalarka\altium export\NUCLEO-F411RE_PCB_BOTTOM_Overlay_Varsay_X_8Dlan_240.ipt
- C:\Users\dvorakj\Documents\Inventor\Bakalarka\altium export\NUCLEO-F411RE_PCB_BOTTOM_Overlay_Varsay_X_8Dlan_241.ipt
- C:\Users\dvorakj\Documents\Inventor\Bakalarka\altium export\NUCLEO-F411RE_PCB_BOTTOM_Overlay_Varsay_X_8Dlan_242.ipt
- C:\Users\dvorakj\Documents\Inventor\Bakalarka\altium export\NUCLEO-F411RE_PCB_BOTTOM_Overlay_Varsay_X_8Dlan_243.ipt
- C:\Users\dvorakj\Documents\Inventor\Bakalarka\altium export\NUCLEO-F411RE_PCB_BOTTOM_Overlay_Varsay_X_8Dlan_244.ipt
- C:\Users\dvorakj\Documents\Inventor\Bakalarka\altium export\NUCLEO-F411RE_PCB_BOTTOM_Overlay_Varsay_X_8Dlan_245.ipt
- C:\Users\dvorakj\Documents\Inventor\Bakalarka\altium export\NUCLEO-F411RE_PCB_BOTTOM_Overlay_Varsay_X_8Dlan_246.ipt
- C:\Users\dvorakj\Documents\Inventor\Bakalarka\altium export\NUCLEO-F411RE_PCB_BOTTOM_Overlay_Varsay_X_8Dlan_247.ipt
- C:\Users\dvorakj\Documents\Inventor\Bakalarka\altium export\NUCLEO-F411RE_PCB_BOTTOM_Overlay_Varsay_X_8Dlan_248.ipt
- C:\Users\dvorakj\Documents\Inventor\Bakalarka\altium export\NUCLEO-F411RE_PCB_BOTTOM_Overlay_Varsay_X_8Dlan_249.ipt
- C:\Users\dvorakj\Documents\Inventor\Bakalarka\altium export\NUCLEO-F411RE_PCB_BOTTOM_Overlay_Varsay_X_8Dlan_250.ipt
- C:\Users\dvorakj\Documents\Inventor\Bakalarka\altium export\NUCLEO-F411RE_PCB_BOTTOM_Overlay_Varsay_X_8Dlan_251.ipt
- C:\Users\dvorakj\Documents\Inventor\Bakalarka\altium export\NUCLEO-F411RE_PCB_BOTTOM_Overlay_Varsay_X_8Dlan_252.ipt
- C:\Users\dvorakj\Documents\Inventor\Bakalarka\altium export\NUCLEO-F411RE_PCB_BOTTOM_Overlay_Varsay_X_8Dlan_253.ipt
- C:\Users\dvorakj\Documents\Inventor\Bakalarka\altium export\NUCLEO-F411RE_PCB_BOTTOM_Overlay_Varsay_X_8Dlan_254.ipt
- C:\Users\dvorakj\Documents\Inventor\Bakalarka\altium export\NUCLEO-F411RE_PCB_BOTTOM_Overlay_Varsay_X_8Dlan_255.ipt
- C:\Users\dvorakj\Documents\Inventor\Bakalarka\altium export\NUCLEO-F411RE_PCB_BOTTOM_Overlay_Varsay_X_8Dlan_256.ipt
- C:\Users\dvorakj\Documents\Inventor\Bakalarka\altium export\NUCLEO-F411RE_PCB_BOTTOM_Overlay_Varsay_X_8Dlan_257.ipt
- C:\Users\dvorakj\Documents\Inventor\Bakalarka\altium export\NUCLEO-F411RE_PCB_BOTTOM_Overlay_Varsay_X_8Dlan_258.ipt
- C:\Users\dvorakj\Documents\Inventor\Bakalarka\altium export\NUCLEO-F411RE_PCB_BOTTOM_Overlay_Varsay_X_8Dlan_259.ipt
- C:\Users\dvorakj\Documents\Inventor\Bakalarka\altium export\NUCLEO-F411RE_PCB_BOTTOM_Overlay_Varsay_X_8Dlan_260.ipt
- C:\Users\dvorakj\Documents\Inventor\Bakalarka\altium export\NUCLEO-F411RE_PCB_BOTTOM_Overlay_Varsay_X_8Dlan_261.ipt
- C:\Users\dvorakj\Documents\Inventor\Bakalarka\altium export\NUCLEO-F411RE_PCB_BOTTOM_Overlay_Varsay_X_8Dlan_262.ipt
- C:\Users\dvorakj\Documents\Inventor\Bakalarka\altium export\NUCLEO-F411RE_PCB_BOTTOM_Overlay_Varsay_X_8Dlan_263.ipt
- C:\Users\dvorakj\Documents\Inventor\Bakalarka\altium export\NUCLEO-F411RE_PCB_BOTTOM_Overlay_Varsay_X_8Dlan_264.ipt
- C:\Users\dvorakj\Documents\Inventor\Bakalarka\altium export\NUCLEO-F411RE_PCB_BOTTOM_Overlay_Varsay_X_8Dlan_265.ipt
- C:\Users\dvorakj\Documents\Inventor\Bakalarka\altium export\NUCLEO-F411RE_PCB_BOTTOM_Overlay_Varsay_X_8Dlan_266.ipt
- C:\Users\dvorakj\Documents\Inventor\Bakalarka\altium export\NUCLEO-F411RE_PCB_BOTTOM_Overlay_Varsay_X_8Dlan_267.ipt
- C:\Users\dvorakj\Documents\Inventor\Bakalarka\altium export\NUCLEO-F411RE_PCB_BOTTOM_Overlay_Varsay_X_8Dlan_268.ipt
- C:\Users\dvorakj\Documents\Inventor\Bakalarka\altium export\NUCLEO-F411RE_PCB_BOTTOM_Overlay_Varsay_X_8Dlan_269.ipt
- C:\Users\dvorakj\Documents\Inventor\Bakalarka\altium export\NUCLEO-F411RE_PCB_BOTTOM_Overlay_Varsay_X_8Dlan_270.ipt
- C:\Users\dvorakj\Documents\Inventor\Bakalarka\altium export\NUCLEO-F411RE_PCB_BOTTOM_Overlay_Varsay_X_8Dlan_271.ipt
- C:\Users\dvorakj\Documents\Inventor\Bakalarka\altium export\NUCLEO-F411RE_PCB_BOTTOM_Overlay_Varsay_X_8Dlan_272.ipt
- C:\Users\dvorakj\Documents\Inventor\Bakalarka\altium export\NUCLEO-F411RE_PCB_BOTTOM_Overlay_Varsay_X_8Dlan_273.ipt
- C:\Users\dvorakj\Documents\Inventor\Bakalarka\altium export\NUCLEO-F411RE_PCB_BOTTOM_Overlay_Varsay_X_8Dlan_274.ipt
- C:\Users\dvorakj\Documents\Inventor\Bakalarka\altium export\NUCLEO-F411RE_PCB_BOTTOM_Overlay_Varsay_X_8Dlan_275.ipt
- C:\Users\dvorakj\Documents\Inventor\Bakalarka\altium export\NUCLEO-F411RE_PCB_BOTTOM_Overlay_Varsay_X_8Dlan_276.ipt
- C:\Users\dvorakj\Documents\Inventor\Bakalarka\altium export\NUCLEO-F411RE_PCB_BOTTOM_Overlay_Varsay_X_8Dlan_277.ipt
- C:\Users\dvorakj\Documents\Inventor\Bakalarka\altium export\NUCLEO-F411RE_PCB_BOTTOM_Overlay_Varsay_X_8Dlan_278.ipt
- C:\Users\dvorakj\Documents\Inventor\Bakalarka\altium export\NUCLEO-F411RE_PCB_BOTTOM_Overlay_Varsay_X_8Dlan_279.ipt
- C:\Users\dvorakj\Documents\Inventor\Bakalarka\altium export\NUCLEO-F411RE_PCB_BOTTOM_Overlay_Varsay_X_8Dlan_280.ipt
- C:\Users\dvorakj\Documents\Inventor\Bakalarka\altium export\NUCLEO-F411RE_PCB_BOTTOM_Overlay_Varsay_X_8Dlan_281.ipt
- C:\Users\dvorakj\Documents\Inventor\Bakalarka\altium export\NUCLEO-F411RE_PCB_BOTTOM_Overlay_Varsay_X_8Dlan_282.ipt
- C:\Users\dvorakj\Documents\Inventor\Bakalarka\altium export\NUCLEO-F411RE_PCB_BOTTOM_Overlay_Varsay_X_8Dlan_283.ipt
- C:\Users\dvorakj\Documents\Inventor\Bakalarka\altium export\NUCLEO-F411RE_PCB_BOTTOM_Overlay_Varsay_X_8Dlan_284.ipt
- C:\Users\dvorakj\Documents\Inventor\Bakalarka\altium export\NUCLEO-F411RE_PCB_BOTTOM_Overlay_Varsay_X_8Dlan_285.ipt
- C:\Users\dvorakj\Documents\Inventor\Bakalarka\altium export\NUCLEO-F411RE_PCB_BOTTOM_Overlay_Varsay_X_8Dlan_286.ipt
- C:\Users\dvorakj\Documents\Inventor\Bakalarka\altium export\NUCLEO-F411RE_PCB_BOTTOM_Overlay_Varsay_X_8Dlan_287.ipt
- C:\Users\dvorakj\Documents\Inventor\Bakalarka\altium export\NUCLEO-F411RE_PCB_BOTTOM_Overlay_Varsay_X_8Dlan_288.ipt
- C:\Users\dvorakj\Documents\Inventor\Bakalarka\altium export\NUCLEO-F411RE_PCB_BOTTOM_Overlay_Varsay_X_8Dlan_289.ipt
- C:\Users\dvorakj\Documents\Inventor\Bakalarka\altium export\NUCLEO-F411RE_PCB_BOTTOM_Overlay_Varsay_X_8Dlan_290.ipt
- C:\Users\dvorakj\Documents\Inventor\Bakalarka\altium export\NUCLEO-F411RE_PCB_BOTTOM_Overlay_Varsay_X_8Dlan_291.ipt
- C:\Users\dvorakj\Documents\Inventor\Bakalarka\altium export\NUCLEO-F411RE_PCB_BOTTOM_Overlay_Varsay_X_8Dlan_292.ipt
- C:\Users\dvorakj\Documents\Inventor\Bakalarka\altium export\NUCLEO-F411RE_PCB_BOTTOM_Overlay_Varsay_X_8Dlan_293.ipt
- C:\Users\dvorakj\Documents\Inventor\Bakalarka\altium export\NUCLEO-F411RE_PCB_BOTTOM_Overlay_Varsay_X_8Dlan_294.ipt
- C:\Users\dvorakj\Documents\Inventor\Bakalarka\altium export\NUCLEO-F411RE_PCB_BOTTOM_Overlay_Varsay_X_8Dlan_295.ipt
- C:\Users\dvorakj\Documents\Inventor\Bakalarka\altium export\NUCLEO-F411RE_PCB_BOTTOM_Overlay_Varsay_X_8Dlan_296.ipt
- C:\Users\dvorakj\Documents\Inventor\Bakalarka\altium export\NUCLEO-F411RE_PCB_BOTTOM_Overlay_Varsay_X_8Dlan_297.ipt
- C:\Users\dvorakj\Documents\Inventor\Bakalarka\altium export\NUCLEO-F411RE_PCB_BOTTOM_Overlay_Varsay_X_8Dlan_298.ipt
- C:\Users\dvorakj\Documents\Inventor\Bakalarka\altium export\NUCLEO-F411RE_PCB_BOTTOM_Overlay_Varsay_X_8Dlan_299.ipt
- C:\Users\dvorakj\Documents\Inventor\Bakalarka\altium export\NUCLEO-F411RE_PCB_BOTTOM_Overlay_Varsay_X_8Dlan_300.ipt
- C:\Users\dvorakj\Documents\Inventor\Bakalarka\altium export\NUCLEO-F411RE_PCB_BOTTOM_Overlay_Varsay_X_8Dlan_301.ipt
- C:\Users\dvorakj\Documents\Inventor\Bakalarka\altium export\NUCLEO-F411RE_PCB_BOTTOM_Overlay_Varsay_X_8Dlan_302.ipt
- C:\Users\dvorakj\Documents\Inventor\Bakalarka\altium export\NUCLEO-F411RE_PCB_BOTTOM_Overlay_Varsay_X_8Dlan_303.ipt
- C:\Users\dvorakj\Documents\Inventor\Bakalarka\altium export\NUCLEO-F411RE_PCB_BOTTOM_Overlay_Varsay_X_8Dlan_304.ipt
- C:\Users\dvorakj\Documents\Inventor\Bakalarka\altium export\NUCLEO-F411RE_PCB_BOTTOM_Overlay_Varsay_X_8Dlan_305.ipt
- C:\Users\dvorakj\Documents\Inventor\Bakalarka\altium export\NUCLEO-F411RE_PCB_BOTTOM_Overlay_Varsay_X_8Dlan_306.ipt
- C:\Users\dvorakj\Documents\Inventor\Bakalarka\altium export\NUCLEO-F411RE_PCB_BOTTOM_Overlay_Varsay_X_8Dlan_307.ipt
- C:\Users\dvorakj\Documents\Inventor\Bakalarka\altium export\NUCLEO-F411RE_PCB_BOTTOM_Overlay_Varsay_X_8Dlan_308.ipt
- C:\Users\dvorakj\Documents\Inventor\Bakalarka\altium export\NUCLEO-F411RE_PCB_BOTTOM_Overlay_Varsay_X_8Dlan_309.ipt
- C:\Users\dvorakj\Documents\Inventor\Bakalarka\altium export\NUCLEO-F411RE_PCB_BOTTOM_Overlay_Varsay_X_8Dlan_310.ipt
- C:\Users\dvorakj\Documents\Inventor\Bakalarka\altium export\NUCLEO-F411RE_PCB_BOTTOM_Overlay_Varsay_X_8Dlan_311.ipt
- C:\Users\dvorakj\Documents\Inventor\Bakalarka\altium export\NUCLEO-F411RE_PCB_BOTTOM_Overlay_Varsay_X_8Dlan_312.ipt
- C:\Users\dvorakj\Documents\Inventor\Bakalarka\altium export\NUCLEO-F411RE_PCB_BOTTOM_Overlay_Varsay_X_8Dlan_313.ipt
- C:\Users\dvorakj\Documents\Inventor\Bakalarka\altium export\NUCLEO-F411RE_PCB_BOTTOM_Overlay_Varsay_X_8Dlan_314.ipt
- C:\Users\dvorakj\Documents\Inventor\Bakalarka\altium export\NUCLEO-F411RE_PCB_BOTTOM_Overlay_Varsay_X_8Dlan_315.ipt
- C:\Users\dvorakj\Documents\Inventor\Bakalarka\altium export\NUCLEO-F411RE_PCB_BOTTOM_Overlay_Varsay_X_8Dlan_316.ipt
- C:\Users\dvorakj\Documents\Inventor\Bakalarka\altium export\NUCLEO-F411RE_PCB_BOTTOM_Overlay_Varsay_X_8Dlan_317.ipt
## Components (318 placed, 318 different names)